# Autodesk Inventor assembly: RT_ARM_A_007_Capstan-Drive
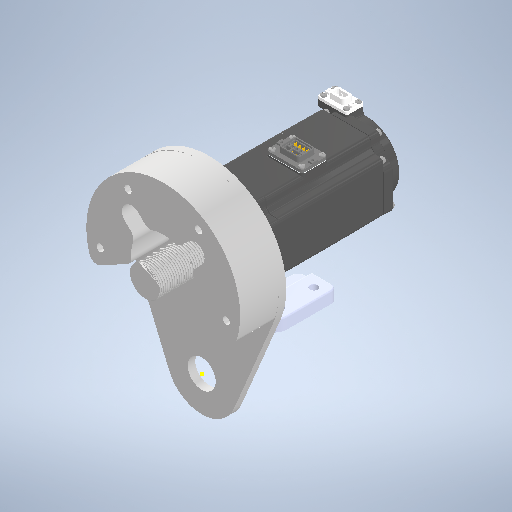
[picture p0: Inventor's stored thumbnail of the model, 512x512]
Saved by Autodesk Inventor 2025.3 (Build 293356000, 356)
## iProperties
Created: 2026-07-28
Part Number: RT_ARM_A_007_Capstan-Drive
Document SubType Name: Assembly
Designer: louis
Author: louis
## Documents named in this file (6)
- C:\Users\louis\OneDrive\Desktop\R_Trident\02_CAD\04_Subassemblies\RT_ARM_A_007_Capstan-Drive.iam
- C:\Users\louis\OneDrive\Desktop\R_Trident\02_CAD\03_Parts_Custom\RT_ARM_MC_008_Capstand_Base.ipt
- C:\Users\louis\OneDrive\Desktop\R_Trident\02_CAD\03_Parts_Custom\RT_ARM_MC_008_Capstand_Support.ipt
- C:\Users\louis\OneDrive\Desktop\R_Trident\02_CAD\01_Standard_Parts\ST-M4\ST-M4.ipt
- C:\Users\louis\OneDrive\Desktop\R_Trident\02_CAD\01_Standard_Parts\A6M60-400H2B1-M17\A6M60-400H2B1-M17.iam
- C:\Users\louis\OneDrive\Desktop\R_Trident\02_CAD\03_Parts_Custom\RT_ARM_PR_008_Capstand_Helical.ipt
## Components (5 placed, 5 different names)
1. RT_ARM_MC_008_Capstand_Base:1 — Flush:1, Flush:2, Flush:3, Mate:1, Mate:2, Mate:3, Mate:4, Mate:6
2. RT_ARM_MC_008_Capstand_Support:1 — Mate:1, Mate:2
3. ST-M4:1 — Mate:3, Mate:4, Mate:5, Mate:8
4. A6M60-400H2B1-M17:1 [sub-assembly] — Mate:6, Mate:7, Mate:8, Mate:9, Mate:10
5. RT_ARM_PR_008_Capstand_Helical:1 — Mate:9, Mate:10
## Relationships (13: Mate 10, Flush 3)
- Flush:1: RT_ARM_MC_008_Capstand_Base:1
- Flush:2: RT_ARM_MC_008_Capstand_Base:1
- Flush:3: RT_ARM_MC_008_Capstand_Base:1
- Mate:1: RT_ARM_MC_008_Capstand_Base:1 ↔ RT_ARM_MC_008_Capstand_Support:1
- Mate:2: RT_ARM_MC_008_Capstand_Base:1 ↔ RT_ARM_MC_008_Capstand_Support:1
- Mate:3: RT_ARM_MC_008_Capstand_Base:1 ↔ ST-M4:1
- Mate:4: RT_ARM_MC_008_Capstand_Base:1 ↔ ST-M4:1
- Mate:5: ST-M4:1
- Mate:6: RT_ARM_MC_008_Capstand_Base:1 ↔ A6M60-400H2B1-M17:1
- Mate:7 (54 mm): A6M60-400H2B1-M17:1
- Mate:8: ST-M4:1 ↔ A6M60-400H2B1-M17:1
- Mate:9: A6M60-400H2B1-M17:1 ↔ RT_ARM_PR_008_Capstand_Helical:1
- Mate:10: A6M60-400H2B1-M17:1 ↔ RT_ARM_PR_008_Capstand_Helical:1
